# Autodesk Inventor assembly: 276-2159
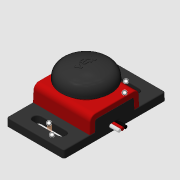
[picture p0: Inventor's stored thumbnail of the model, 180x180]
Saved by Autodesk Inventor 2021 (Build 250183000, 183)
## iProperties
Part Number: 276-2159
Document SubType Name: Assembly
Designer: Jordan Kiesel
Mass: 19.051 g
Surface Area: 118.61 cm^2
Volume: 8.27156 cm^3
Density: 2.30319 g/cm^3
Catalog Web Link: vexrobotics.com/276-2159.html
Description: Useful as a trigger in a variety of applications.
Vendor: VEX Robotics, Inc.
Created: 2020-04-23
Category: Sensors
Company: Super Sonic Sparks, Team 24
Translation Standard: STEP AP203
FileName: Bumper Switch.iam
PreProcessor: SolidWorks 2006052
PostProcessor: Build: 239, Release: 2011 RTM - Date: Wed 02/17/2010
Sent Units: inch
Uncertainty: 1e-05
Author: Jordan Kiesel
Title: Bumper Switch
Comments: Simple bumper switch custom built for the VEX Robotics Design System. Ruggedized Bumpers allow the switch to be triggered by large impacts without sustaining damage. ▷ Provide feedback to Microcontroller as events "happen". ▷ Rugged bumper allows switch to be triggered without damage. ▷ Useful as a trigger in a variety of applications. ▷ Functionality is pre-programmed in the VEX Microcontroller.
## Documents named in this file (6)
- E:\2020 BNS-VRC-SID-YY Library\Electronics\Sensors\Bumper Switch.iam
- E:\2020 BNS-VRC-SID-YY Library\Electronics\Sensors\Reference Parts\Bumper Switch\Top.ipt
- E:\2020 BNS-VRC-SID-YY Library\Electronics\Sensors\Reference Parts\Bumper Switch\Bottom.ipt
- E:\2020 BNS-VRC-SID-YY Library\Electronics\Sensors\Reference Parts\Bumper Switch\Inner Head.ipt
- E:\2020 BNS-VRC-SID-YY Library\Electronics\Sensors\Reference Parts\Bumper Switch\Head.ipt
- E:\2020 BNS-VRC-SID-YY Library\Electronics\Sensors\Reference Parts\Sensors\3-Wire Black-Red-White Cable, Cut.ipt
## Components (5 placed, 5 different names)
1. Top:1 — Insert:2, Insert:3, Insert:4, Angle:3
2. Bottom:1 — Angle:1, Insert:3, Insert:4, Tangent:1, Tangent:2, Angle:2, Tangent:3
3. Inner Head:1 — Insert:1, Insert:2, Angle:3
4. Head:1 — Insert:1, Angle:1
5. 3-Wire Black-Red-White Cable, Cut:1 — Tangent:1, Tangent:2, Angle:2, Tangent:3
## Relationships (10: Insert 4, Angle 3, Tangent 3)
- Insert:1: Inner Head:1 ↔ Head:1
- Angle:1 (0 deg): Bottom:1 ↔ Head:1
- Insert:2 (2.6924 mm): Top:1 ↔ Inner Head:1
- Insert:3: Top:1 ↔ Bottom:1
- Insert:4: Top:1 ↔ Bottom:1
- Tangent:1 (0.6477 mm): Bottom:1 ↔ 3-Wire Black-Red-White Cable, Cut:1
- Tangent:2 (0.889 mm): Bottom:1 ↔ 3-Wire Black-Red-White Cable, Cut:1
- Angle:2 (0 deg): Bottom:1 ↔ 3-Wire Black-Red-White Cable, Cut:1
- Tangent:3 (0.889 mm): Bottom:1 ↔ 3-Wire Black-Red-White Cable, Cut:1
- Angle:3 (-40 deg): Top:1 ↔ Inner Head:1
